# Autodesk Inventor assembly: wheel_drive_kit
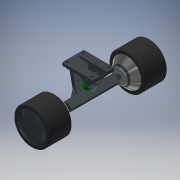
[picture p0: Inventor's stored thumbnail of the model, 180x180]
Saved by Autodesk Inventor 2017 SP1 (Build 210196100, 196)
## iProperties
Part Number: wheel_drive_kit
Material: 一般
Document SubType Name: Assembly
Designer: gisen
Author: gisen
## Documents named in this file (4)
- C:\Users\gisen\Documents\myElectricSk8\CAD\wheel_drive_kit.iam
- C:\Users\gisen\Documents\myElectricSk8\CAD\shaft_drive.ipt
- C:\Users\gisen\Documents\myElectricSk8\CAD\wheel_drive.ipt
- C:\Users\gisen\Documents\myElectricSk8\CAD\shaft_jig.ipt
## Components (4 placed, 3 different names)
1. shaft_drive:1 — メイト:2, メイト:3, メイト:4, メイト:5, メイト:6, メイト:7, メイト:8
2. wheel_drive:1 — メイト:7, メイト:8
3. wheel_drive:2 — メイト:5, メイト:6
4. shaft_jig:1 — フラッシュ:1, メイト:1, フラッシュ:2, メイト:2, メイト:3, メイト:4
## Relationships (10: Mate 8, Flush 2)
- フラッシュ:1 [Flush]: shaft_jig:1
- メイト:1 [Mate]: shaft_jig:1
- フラッシュ:2 [Flush]: shaft_jig:1
- メイト:2 [Mate]: shaft_drive:1 ↔ shaft_jig:1
- メイト:3 [Mate]: shaft_drive:1 ↔ shaft_jig:1
- メイト:4 [Mate]: shaft_drive:1 ↔ shaft_jig:1
- メイト:5 [Mate]: shaft_drive:1 ↔ wheel_drive:2
- メイト:6 [Mate]: shaft_drive:1 ↔ wheel_drive:2
- メイト:7 [Mate]: shaft_drive:1 ↔ wheel_drive:1
- メイト:8 [Mate]: shaft_drive:1 ↔ wheel_drive:1
